# Autodesk Inventor assembly: JF_0837B_Linear solenoid Pull 15N 12v1A
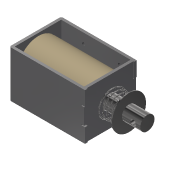
[picture p0: Inventor's stored thumbnail of the model, 180x180]
Saved by Autodesk Inventor 2018.3 (Build 223284000, 284)
## iProperties
Manager: GURSKY
Company: ltd "MRF-ENGINEERING"
Created: 2017-09-28
Part Number: JF_0837B_Linear solenoid Pull 15N 12v1A
Project: 1708
Checked By: Гурский
Engr Approved By: ---
Catalog Web Link: http://en.solenoid-bs.com/products_detail/productId=43.html
Vendor: ltd "MRF-ENGINEERING"
Document SubType Name: Assembly
Designer: Макс
Engineer: TIHONOV
Authority: GURSKY
Stock Number: BS-1684-01
Description: Linear solenoid push pull type
Title: Linear solenoid push pull type
Subject: Filling machine
Author: Макс
## Documents named in this file (4)
- C:\Vault\Projects\Imported Components\BS-1684-01_Linear solenoid\JF_0837B_Linear solenoid Pull 15N 12v1A.iam
- C:\Vault\Projects\Imported Components\BS-1684-01_Linear solenoid\BS-1684-01_Linear solenoid push pull type_Frame.ipt
- C:\Vault\Projects\Imported Components\BS-1684-01_Linear solenoid\BS-1684-01_Linear solenoid push pull type_SHTOK.ipt
- C:\Vault\Projects\Imported Components\BS-1684-01_Linear solenoid\BS-1684-01_Linear solenoid push pull type_spring.ipt
## Components (3 placed, 3 different names)
1. BS-1684-01_Linear solenoid push pull type_Frame:1 — Совмещение:1, Совмещение:2, Заподлицо:3
2. BS-1684-01_Linear solenoid push pull type_SHTOK:1 — Совмещение:1, Совмещение:2, Угол:1, Совмещение:5
3. BS-1684-01_Linear solenoid push pull type_spring:1 — Заподлицо:3, Совмещение:5
## Relationships (5: Mate 3, Angle 1, Flush 1)
- Совмещение:1 [Mate]: BS-1684-01_Linear solenoid push pull type_Frame:1 ↔ BS-1684-01_Linear solenoid push pull type_SHTOK:1
- Совмещение:2 [Mate]: BS-1684-01_Linear solenoid push pull type_Frame:1 ↔ BS-1684-01_Linear solenoid push pull type_SHTOK:1
- Угол:1 [Angle] (180 deg): BS-1684-01_Linear solenoid push pull type_SHTOK:1
- Заподлицо:3 [Flush]: BS-1684-01_Linear solenoid push pull type_Frame:1 ↔ BS-1684-01_Linear solenoid push pull type_spring:1
- Совмещение:5 [Mate]: BS-1684-01_Linear solenoid push pull type_SHTOK:1 ↔ BS-1684-01_Linear solenoid push pull type_spring:1
